# Autodesk Inventor assembly: fullWrench
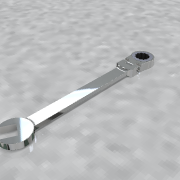
[picture p0: Inventor's stored thumbnail of the model, 180x180]
Saved by Autodesk Inventor 2017 (Build 210142000, 142)
## iProperties
Created: 2017-02-16
Part Number: fullWrench
Document SubType Name: Assembly
Designer: kingb
Author: kingb
## Documents named in this file (4)
- C:\Users\kingb\Desktop\CAD\fullWrench.iam
- C:\Users\kingb\Desktop\CAD\wrenchA.ipt
- C:\Users\kingb\Desktop\CAD\wrenchB.ipt
- C:\Users\kingb\Desktop\CAD\wrenchC.ipt
## Components (3 placed, 3 different names)
1. wrenchA:1 — Flush:1, Mate:1, Mate:2, Angle:1
2. wrenchB:1 — Flush:1, Mate:1, Mate:2, Angle:1, Flush:2, Flush:3
3. wrenchC:1 — Flush:2, Flush:3
## Relationships (6: Flush 3, Mate 2, Angle 1)
- Flush:1: wrenchA:1 ↔ wrenchB:1
- Mate:1: wrenchA:1 ↔ wrenchB:1
- Mate:2: wrenchA:1 ↔ wrenchB:1
- Angle:1 (0 deg): wrenchA:1 ↔ wrenchB:1
- Flush:2: wrenchB:1 ↔ wrenchC:1
- Flush:3: wrenchB:1 ↔ wrenchC:1
